# Autodesk Inventor assembly: 足全体_MIR
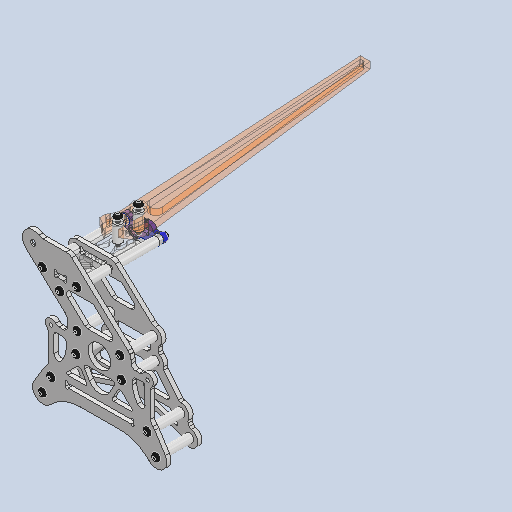
[picture p0: Inventor's stored thumbnail of the model, 512x512]
Saved by Autodesk Inventor 2023.1 (Build 271208000, 208)
## iProperties
Created: 2022-01-30
Part Number: 足全体_MIR
Document SubType Name: Assembly
Designer: muzho
Mass: 81.1027 g
Surface Area: 503.794 cm^2
Volume: 45.5138 cm^3
Density: 1.78194 g/cm^3
Author: acps
## Documents named in this file (14)
- C:\Users\muzho\Documents\srdc\srdc_2\脚\MIR\中間ユニット_MIR.iam
- C:\Users\muzho\Documents\srdc\srdc_2\脚\ウィング関連\MIR\足 横wing下板 _MIR.ipt
- C:\Users\muzho\Documents\srdc\srdc_2\脚\ウィング関連\MIR\足 横wing固定用外フレーム_MIR.ipt
- C:\Users\muzho\Documents\srdc\srdc_2\脚\ウィング関連\MIR\横wing 押さえ_MIR.ipt
- C:\Users\muzho\Documents\srdc\srdc_2\脚\ウィング関連\MIR\横wing _MIR_MIR.ipt
- C:\Users\muzho\Documents\srdc\srdc_2\脚\MIR\外中間ユニット_MIR.ipt
- C:\Users\muzho\Documents\srdc\srdc_2\脚\MIR\内中間ユニット_MIR.ipt
- C:\Users\muzho\Documents\srdc\srdc_2\スペーサ\l3.ipt
- C:\Users\muzho\Documents\srdc\srdc_2\スペーサ\l30.ipt
- C:\Users\muzho\Documents\srdc\srdc_2\スペーサ\l23_peak.ipt
- C:\Users\muzho\Documents\srdc\srdc_2\スペーサ\l12.ipt
- C:\Users\muzho\Documents\srdc\srdc_2\ねじ\M3ボタンボルト18.ipt
- C:\Users\muzho\Documents\srdc\srdc_2\スペーサ\l23.ipt
- C:\Users\muzho\Documents\srdc\srdc_2\ねじ\M3ボタンボルト8.ipt
## Components (49 placed, 13 different names)
1. 足 横wing下板 _MIR:1 — メイト:17, フラッシュ:1, メイト:23, メイト:22, 挿入:10, 挿入:11
2. 足 横wing固定用外フレーム_MIR:1 — 挿入:2, 挿入:5, 挿入:6, 挿入:32, 挿入:33, 挿入:34
3. 横wing 押さえ_MIR:1 — 挿入:12, 挿入:13, 挿入:14, 挿入:15
4. 横wing _MIR_MIR:1 — メイト:17, メイト:5, メイト:6
5. 外中間ユニット_MIR:1 — メイト:21, 挿入:7, 挿入:16, 挿入:17, 挿入:18, 挿入:19, 挿入:20, 挿入:21, 挿入:22, 挿入:23, 挿入:35, 挿入:36, 挿入:37, 挿入:39, 挿入:40, 挿入:41, 挿入:42, 挿入:43, 挿入:44, 挿入:45, 挿入:50
6. 内中間ユニット_MIR:1 — フラッシュ:1, メイト:23, メイト:22, メイト:21, 挿入:24, 挿入:25, 挿入:26, 挿入:27, 挿入:28, 挿入:29, 挿入:30, 挿入:31, 挿入:46, 挿入:47, 挿入:48, 挿入:49
7. l3:1 — 挿入:2
8. l30:1 — 挿入:45
9. l3:2 — 挿入:5
10. l30:2 — 挿入:44
11. l3:3 — 挿入:6
12. l30:3
13. l23_peak:1 — 挿入:7
14. l23_peak:2 — 挿入:50
15. l23_peak:3
16. l12:1 — 挿入:11, 挿入:13, メイト:6
17. l12:2 — 挿入:10, 挿入:12, メイト:5
18. M3ボタンボルト18:1 — 挿入:14
19. M3ボタンボルト18:2 — 挿入:15
20. l23:1 — 挿入:21
21. l23:2 — 挿入:20
22. l23:3 — 挿入:16
23. l23:4 — 挿入:17
24. l23:5 — 挿入:19
25. l23:6 — 挿入:18, 挿入:49
26. l23:7 — 挿入:22
27. l23:8 — 挿入:23
28. M3ボタンボルト8:1 — 挿入:30
29. M3ボタンボルト8:2 — 挿入:27
30. M3ボタンボルト8:3 — 挿入:28
31. M3ボタンボルト8:5 — 挿入:34
32. M3ボタンボルト8:6 — 挿入:35
33. M3ボタンボルト8:7 — 挿入:31
34. M3ボタンボルト8:8 — 挿入:32
35. M3ボタンボルト8:9 — 挿入:33
36. M3ボタンボルト8:10 — 挿入:29
37. M3ボタンボルト8:11 — 挿入:24
38. M3ボタンボルト8:12 — 挿入:26
39. M3ボタンボルト8:13 — 挿入:25
40. M3ボタンボルト8:14 — 挿入:37
41. M3ボタンボルト8:15 — 挿入:40
42. M3ボタンボルト8:16 — 挿入:39
43. M3ボタンボルト8:17 — 挿入:43
44. M3ボタンボルト8:18 — 挿入:42
45. M3ボタンボルト8:19 — 挿入:41
46. M3ボタンボルト8:21 — 挿入:36
47. M3ボタンボルト8:22 — 挿入:46
48. M3ボタンボルト8:23 — 挿入:47
49. M3ボタンボルト8:24 — 挿入:48
## Relationships (54: Insert 47, Mate 6, Flush 1)
- メイト:17 [Mate] (5 mm): 足 横wing下板 _MIR:1 ↔ 横wing _MIR_MIR:1
- フラッシュ:1 [Flush]: 足 横wing下板 _MIR:1 ↔ 内中間ユニット_MIR:1
- メイト:23 [Mate]: 足 横wing下板 _MIR:1 ↔ 内中間ユニット_MIR:1
- メイト:22 [Mate]: 足 横wing下板 _MIR:1 ↔ 内中間ユニット_MIR:1
- メイト:21 [Mate]: 外中間ユニット_MIR:1 ↔ 内中間ユニット_MIR:1
- [Insert]: l3:1 ↔ l30:1
- 挿入:2 [Insert]: 足 横wing固定用外フレーム_MIR:1 ↔ l3:1
- [Insert]: l3:2 ↔ l30:2
- [Insert]: l3:3 ↔ l30:3
- 挿入:5 [Insert]: 足 横wing固定用外フレーム_MIR:1 ↔ l3:2
- 挿入:6 [Insert]: 足 横wing固定用外フレーム_MIR:1 ↔ l3:3
- 挿入:7 [Insert]: 外中間ユニット_MIR:1 ↔ l23_peak:1
- 挿入:10 [Insert]: 足 横wing下板 _MIR:1 ↔ l12:2
- 挿入:11 [Insert]: 足 横wing下板 _MIR:1 ↔ l12:1
- 挿入:12 [Insert]: 横wing 押さえ_MIR:1 ↔ l12:2
- 挿入:13 [Insert]: 横wing 押さえ_MIR:1 ↔ l12:1
- 挿入:14 [Insert]: 横wing 押さえ_MIR:1 ↔ M3ボタンボルト18:1
- 挿入:15 [Insert]: 横wing 押さえ_MIR:1 ↔ M3ボタンボルト18:2
- 挿入:16 [Insert]: 外中間ユニット_MIR:1 ↔ l23:3
- 挿入:17 [Insert]: 外中間ユニット_MIR:1 ↔ l23:4
- 挿入:18 [Insert]: 外中間ユニット_MIR:1 ↔ l23:6
- 挿入:19 [Insert]: 外中間ユニット_MIR:1 ↔ l23:5
- 挿入:20 [Insert]: 外中間ユニット_MIR:1 ↔ l23:2
- 挿入:21 [Insert]: 外中間ユニット_MIR:1 ↔ l23:1
- 挿入:22 [Insert]: 外中間ユニット_MIR:1 ↔ l23:7
- 挿入:23 [Insert]: 外中間ユニット_MIR:1 ↔ l23:8
- 挿入:24 [Insert]: 内中間ユニット_MIR:1 ↔ M3ボタンボルト8:11
- 挿入:25 [Insert]: 内中間ユニット_MIR:1 ↔ M3ボタンボルト8:13
- 挿入:26 [Insert]: 内中間ユニット_MIR:1 ↔ M3ボタンボルト8:12
- 挿入:27 [Insert]: 内中間ユニット_MIR:1 ↔ M3ボタンボルト8:2
- 挿入:28 [Insert]: 内中間ユニット_MIR:1 ↔ M3ボタンボルト8:3
- 挿入:29 [Insert]: 内中間ユニット_MIR:1 ↔ M3ボタンボルト8:10
- 挿入:30 [Insert]: 内中間ユニット_MIR:1 ↔ M3ボタンボルト8:1
- 挿入:31 [Insert]: 内中間ユニット_MIR:1 ↔ M3ボタンボルト8:7
- 挿入:32 [Insert]: 足 横wing固定用外フレーム_MIR:1 ↔ M3ボタンボルト8:8
- 挿入:33 [Insert]: 足 横wing固定用外フレーム_MIR:1 ↔ M3ボタンボルト8:9
- 挿入:34 [Insert]: 足 横wing固定用外フレーム_MIR:1 ↔ M3ボタンボルト8:5
- 挿入:35 [Insert]: 外中間ユニット_MIR:1 ↔ M3ボタンボルト8:6
- 挿入:36 [Insert]: 外中間ユニット_MIR:1 ↔ M3ボタンボルト8:21
- 挿入:37 [Insert]: 外中間ユニット_MIR:1 ↔ M3ボタンボルト8:14
- 挿入:39 [Insert]: 外中間ユニット_MIR:1 ↔ M3ボタンボルト8:16
- 挿入:40 [Insert]: 外中間ユニット_MIR:1 ↔ M3ボタンボルト8:15
- 挿入:41 [Insert]: 外中間ユニット_MIR:1 ↔ M3ボタンボルト8:19
- 挿入:42 [Insert]: 外中間ユニット_MIR:1 ↔ M3ボタンボルト8:18
- 挿入:43 [Insert]: 外中間ユニット_MIR:1 ↔ M3ボタンボルト8:17
- 挿入:44 [Insert]: 外中間ユニット_MIR:1 ↔ l30:2
- 挿入:45 [Insert]: 外中間ユニット_MIR:1 ↔ l30:1
- メイト:5 [Mate]: 横wing _MIR_MIR:1 ↔ l12:2
- メイト:6 [Mate]: 横wing _MIR_MIR:1 ↔ l12:1
- 挿入:46 [Insert]: 内中間ユニット_MIR:1 ↔ M3ボタンボルト8:22
- 挿入:47 [Insert]: 内中間ユニット_MIR:1 ↔ M3ボタンボルト8:23
- 挿入:48 [Insert]: 内中間ユニット_MIR:1 ↔ M3ボタンボルト8:24
- 挿入:49 [Insert]: 内中間ユニット_MIR:1 ↔ l23:6
- 挿入:50 [Insert]: 外中間ユニット_MIR:1 ↔ l23_peak:2
## Named parameters: d7_d113 = 0 mm, d8_d113 = 0 mm
